# Autodesk Inventor assembly: Full Assembly-2
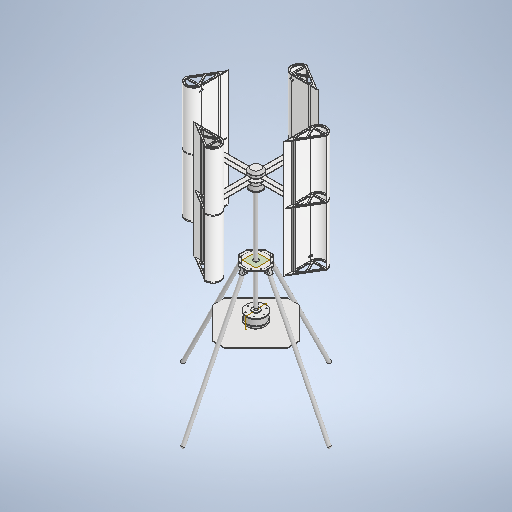
[picture p0: Inventor's stored thumbnail of the model, 512x512]
Saved by Autodesk Inventor 2025.1 (Build 291241000, 241)
## iProperties
Created: 2025-01-28
Part Number: Full Assembly-2
Document SubType Name: Assembly
Designer: Dimas Arif
Author: Dimas Arif
## Documents named in this file (6)
- C:\Users\Dimas Arif\Documents\Inventor\Project-81\Full Assembly-2.iam
- C:\Users\Dimas Arif\Documents\Inventor\Project-81\Blade.iam
- C:\Users\Dimas Arif\Documents\Inventor\Project-81\H1.ipt
- C:\Users\Dimas Arif\Documents\Inventor\Project-81\Motor.ipt
- C:\Users\Dimas Arif\Documents\Inventor\Content Center Files\R2025\en-US\ISO 4762(2)\ISO 4762 - M8 x 20ISO.ipt
- C:\Users\Dimas Arif\Documents\Inventor\Content Center Files\R2025\en-US\ISO 4032(2)\ISO 4032 - M8 - ISO.ipt
## Components (19 placed, 5 different names)
1. Blade:1 [sub-assembly] — Mate:1, Mate:2, Flush:1
2. H1:1 — Mate:1, Mate:2, Flush:1, Mate:3, Mate:4, Mate:5, Mate:6, Mate:7, Mate:8, Mate:9, Mate:10, Mate:11, Mate:12, Mate:13, Mate:14, Mate:15, Mate:16, Mate:17, Mate:18, Mate:19, Mate:20, Insert:1, Insert:2, Insert:3, Insert:4, Insert:5, Insert:6, Insert:7, Insert:8
3. Motor:1 — Mate:3, Mate:4
4. ISO 4762 M8 x 20:1 — Mate:5, Mate:6
5. ISO 4762 M8 x 20:2 — Mate:7, Mate:8
6. ISO 4762 M8 x 20:3 — Mate:9, Mate:10
7. ISO 4762 M8 x 20:4 — Mate:11, Mate:12
8. ISO 4762 M8 x 20:5 — Mate:13, Mate:14
9. ISO 4762 M8 x 20:6 — Mate:15, Mate:16
10. ISO 4762 M8 x 20:7 — Mate:17, Mate:18
11. ISO 4762 M8 x 20:8 — Mate:19, Mate:20
12. ISO 4032 M8:1 — Insert:1
13. ISO 4032 M8:2 — Insert:2
14. ISO 4032 M8:3 — Insert:3
15. ISO 4032 M8:4 — Insert:4
16. ISO 4032 M8:5 — Insert:5
17. ISO 4032 M8:6 — Insert:6
18. ISO 4032 M8:7 — Insert:7
19. ISO 4032 M8:8 — Insert:8
## Relationships (29: Mate 20, Insert 8, Flush 1)
- Mate:1: Blade:1 ↔ H1:1
- Mate:2: Blade:1 ↔ H1:1
- Flush:1: Blade:1 ↔ H1:1
- Mate:3: H1:1 ↔ Motor:1
- Mate:4: H1:1 ↔ Motor:1
- Mate:5: H1:1 ↔ ISO 4762 M8 x 20:1
- Mate:6: H1:1 ↔ ISO 4762 M8 x 20:1
- Mate:7: H1:1 ↔ ISO 4762 M8 x 20:2
- Mate:8: H1:1 ↔ ISO 4762 M8 x 20:2
- Mate:9: H1:1 ↔ ISO 4762 M8 x 20:3
- Mate:10: H1:1 ↔ ISO 4762 M8 x 20:3
- Mate:11: H1:1 ↔ ISO 4762 M8 x 20:4
- Mate:12: H1:1 ↔ ISO 4762 M8 x 20:4
- Mate:13: H1:1 ↔ ISO 4762 M8 x 20:5
- Mate:14: H1:1 ↔ ISO 4762 M8 x 20:5
- Mate:15: H1:1 ↔ ISO 4762 M8 x 20:6
- Mate:16: H1:1 ↔ ISO 4762 M8 x 20:6
- Mate:17: H1:1 ↔ ISO 4762 M8 x 20:7
- Mate:18: H1:1 ↔ ISO 4762 M8 x 20:7
- Mate:19: H1:1 ↔ ISO 4762 M8 x 20:8
- Mate:20: H1:1 ↔ ISO 4762 M8 x 20:8
- Insert:1: H1:1 ↔ ISO 4032 M8:1
- Insert:2: H1:1 ↔ ISO 4032 M8:2
- Insert:3: H1:1 ↔ ISO 4032 M8:3
- Insert:4: H1:1 ↔ ISO 4032 M8:4
- Insert:5: H1:1 ↔ ISO 4032 M8:5
- Insert:6: H1:1 ↔ ISO 4032 M8:6
- Insert:7: H1:1 ↔ ISO 4032 M8:7
- Insert:8: H1:1 ↔ ISO 4032 M8:8
